# Autodesk Inventor assembly: ASY МОО 001 отстойник осветлитель
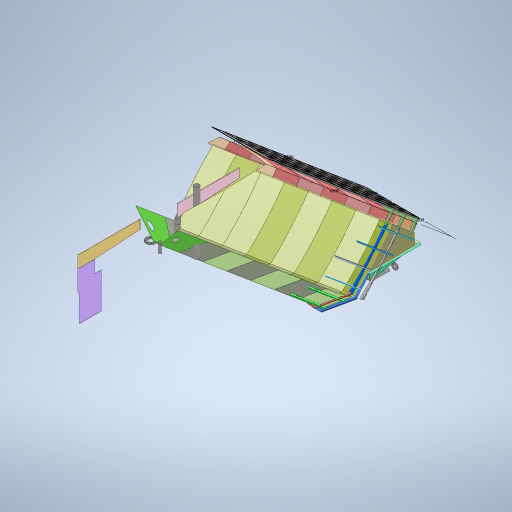
[picture p0: Inventor's stored thumbnail of the model, 512x512]
Saved by Autodesk Inventor 2024.2 (Build 282272000, 272)
## iProperties
Created: 2024-04-28
Part Number: ASY МОО 001 отстойник осветлитель
Document SubType Name: Weldment
Designer: admin
Weld Material: Welded Aluminum-6061
Mass: 1.58517e+06 g
Surface Area: 1.48953e+06 cm^2
Volume: 226523 cm^3
Density: 6.99781 g/cm^3
Author: admin
## Documents named in this file (42)
- C:\Users\admin\YandexDisk-badmisterfox\домашниий пк\Inventor\Manturovo\Manturovo_Se-clar\ASY МОО 001 отстойник осветлитель.iam
- C:\Users\admin\YandexDisk-badmisterfox\домашниий пк\Inventor\Manturovo\Manturovo_Se-clar\МОО 010 лист спина 1.ipt
- C:\Users\admin\YandexDisk-badmisterfox\домашниий пк\Inventor\Manturovo\Manturovo_Se-clar\Пример емкости.ipt
- C:\Users\admin\YandexDisk-badmisterfox\домашниий пк\Inventor\Manturovo\Manturovo_Se-clar\МОО 030 лист брюхо 1.ipt
- C:\Users\admin\YandexDisk-badmisterfox\домашниий пк\Inventor\Manturovo\Manturovo_Se-clar\МОО 040 шпангоут борт 1.ipt
- C:\Users\admin\YandexDisk-badmisterfox\домашниий пк\Inventor\Manturovo\Manturovo_Se-clar\МОО 041 шпангоут спина 1.ipt
- C:\Users\admin\YandexDisk-badmisterfox\домашниий пк\Inventor\Manturovo\Manturovo_Se-clar\Рама основания\ASY МОО 040 рама основания.iam
- C:\Users\admin\YandexDisk-badmisterfox\домашниий пк\Inventor\Manturovo\Manturovo_Se-clar\ASY МОО 060 ракета.iam
- C:\Users\admin\YandexDisk-badmisterfox\домашниий пк\Inventor\Manturovo\Manturovo_Se-clar\Content Center Files\en-US\ISO 5251 B 3D\ISO 5251 Bends 3D without straight ends(90 deg) DN80 2 2.ipt
- C:\Users\admin\YandexDisk-badmisterfox\домашниий пк\Inventor\Manturovo\Manturovo_Se-clar\Content Center Files\en-US\ISO 5251(1)\ISO 5251 Concentric reducers DN80 x DN65 3,2 3,2.ipt
- C:\Users\admin\YandexDisk-badmisterfox\домашниий пк\Inventor\Manturovo\Manturovo_Se-clar\ASY МОО 020 конус.iam
- C:\Users\admin\YandexDisk-badmisterfox\домашниий пк\Inventor\Manturovo\Manturovo_Se-clar\ракета\МОО 064 ракета труба.ipt
- C:\Users\admin\YandexDisk-badmisterfox\домашниий пк\Inventor\Manturovo\Manturovo_Se-clar\х_размеры МОО отстойник осветлитель Dummu.ipt
- C:\Users\admin\YandexDisk-badmisterfox\домашниий пк\Inventor\Manturovo\Manturovo_Se-clar\МОО 012 лист спина 2.ipt
- C:\Users\admin\YandexDisk-badmisterfox\домашниий пк\Inventor\Manturovo\Manturovo_Se-clar\Content Center Files\en-US\DIN EN 1092-1 01 - PN 25\DIN EN 1092-1 Plate Flange for Welding Type 01 - PN 25 80 x 88.9.ipt
- C:\Users\admin\YandexDisk-badmisterfox\домашниий пк\Inventor\Manturovo\Manturovo_Se-clar\МОО 011 лист борт.ipt
- C:\Users\admin\YandexDisk-badmisterfox\домашниий пк\Inventor\Manturovo\Manturovo_Se-clar\МОО 010 лист спина-бедро.ipt
- C:\Users\admin\YandexDisk-badmisterfox\домашниий пк\Inventor\Manturovo\Manturovo_Se-clar\МОО 011 лист борт левый борт бедро.ipt
- C:\Users\admin\YandexDisk-badmisterfox\домашниий пк\Inventor\Manturovo\Manturovo_Se-clar\МОО 011 лист борт правый борт бедро.ipt
- C:\Users\admin\YandexDisk-badmisterfox\домашниий пк\Inventor\Manturovo\Manturovo_Se-clar\МОО 014 лист спина-холка.ipt
- C:\Users\admin\YandexDisk-badmisterfox\домашниий пк\Inventor\Manturovo\Manturovo_Se-clar\МОО 032 лист брюхо-горло.ipt
- C:\Users\admin\YandexDisk-badmisterfox\домашниий пк\Inventor\Manturovo\Manturovo_Se-clar\МОО 035 лист борт.ipt
- C:\Users\admin\YandexDisk-badmisterfox\домашниий пк\Inventor\Manturovo\Manturovo_Se-clar\конус\МОО 051 гребень 1.ipt
- C:\Users\admin\YandexDisk-badmisterfox\домашниий пк\Inventor\Manturovo\Manturovo_Se-clar\конус\МОО 052 гребень 2.ipt
- C:\Users\admin\YandexDisk-badmisterfox\домашниий пк\Inventor\Manturovo\Manturovo_Se-clar\конус\МОО 053 морда 3.ipt
- C:\Users\admin\YandexDisk-badmisterfox\домашниий пк\Inventor\Manturovo\Manturovo_Se-clar\Content Center Files\en-US\ISO 5251 B 3D\ISO 5251 Bends 3D without straight ends(90 deg) DN150 11 11.ipt
- C:\Users\admin\YandexDisk-badmisterfox\домашниий пк\Inventor\Manturovo\Manturovo_Se-clar\Content Center Files\en-US\DIN EN 1092-1 01 - PN 25\DIN EN 1092-1 Plate Flange for Welding Type 01 - PN 25 150 x 168.3.ipt
- C:\Users\admin\YandexDisk-badmisterfox\домашниий пк\Inventor\Manturovo\Manturovo_Se-clar\МОО 061 труба верх 1.ipt
- C:\Users\admin\YandexDisk-badmisterfox\домашниий пк\Inventor\Manturovo\Manturovo_Se-clar\МОО 062 труба верх 2.ipt
- C:\Users\admin\YandexDisk-badmisterfox\домашниий пк\Inventor\Manturovo\Manturovo_Se-clar\МОО 063 труба верх 3.ipt
- C:\Users\admin\YandexDisk-badmisterfox\домашниий пк\Inventor\Manturovo\Manturovo_Se-clar\МОО 051 стрингер спина 1.ipt
- C:\Users\admin\YandexDisk-badmisterfox\домашниий пк\Inventor\Manturovo\Manturovo_Se-clar\МОО 053 стрингер борт 3.ipt
- C:\Users\admin\YandexDisk-badmisterfox\домашниий пк\Inventor\Manturovo\Manturovo_Se-clar\МОО 052 стрингер спина 22.ipt
- C:\Users\admin\YandexDisk-badmisterfox\домашниий пк\Inventor\Manturovo\Manturovo_Se-clar\МОО 054 стрингер борт 43.ipt
- C:\Users\admin\YandexDisk-badmisterfox\домашниий пк\Inventor\Manturovo\Manturovo_Se-clar\МОО 055 стрингер борт 52.ipt
- C:\Users\admin\YandexDisk-badmisterfox\домашниий пк\Inventor\Manturovo\Manturovo_Se-clar\МОО 056 стрингер борт 62.ipt
- C:\Users\admin\YandexDisk-badmisterfox\домашниий пк\Inventor\Manturovo\Manturovo_Se-clar\МОО 057 стрингер борт 7.ipt
- C:\Users\admin\YandexDisk-badmisterfox\домашниий пк\Inventor\Manturovo\Manturovo_Se-clar\МОО 042 шпангоут брюхо.ipt
- C:\Users\admin\YandexDisk-badmisterfox\домашниий пк\Inventor\Manturovo\Manturovo_Se-clar\МОО 025 лист борт холка.ipt
- C:\Users\admin\YandexDisk-badmisterfox\домашниий пк\Inventor\Manturovo\Manturovo_Se-clar\МОО 026 лист борт морда.ipt
- C:\Users\admin\YandexDisk-badmisterfox\домашниий пк\Inventor\Manturovo\Manturovo_Se-clar\Part1.ipt
- C:\Users\admin\YandexDisk-badmisterfox\домашниий пк\Inventor\Manturovo\Manturovo_Se-clar\стапель\ASY стапель.iam
## Components (82 placed, 43 different names)
1. Пример емкости:1 — Mate:1, Mate:2, Flush:2
2. х_размеры МОО отстойник осветлитель Dummu:1
3. ASY МОО 040 рама основания:1 [sub-assembly] — Flush:19, Flush:20, Flush:21
4. МОО 010 лист спина 1:1 — Flush:3, Rigid:11, Rigid:12
5. МОО 030 лист брюхо 1:1 — Mate:9, Rigid:18, Rigid:40
6. ASY МОО 060 ракета:1 [sub-assembly] — Flush:23, Rigid:10
7. ISO 5251 Bends 3D without straight ends(90 deg) DN80 2:1 — Rigid:2, Rigid:3
8. ISO 5251 Concentric reducers DN80 x DN65 3,2:1 — Rigid:2, Rigid:10
9. ASY МОО 020 конус:1 [sub-assembly] — Flush:22, Mate:16, Flush:28, Mate:31, Mate:36, Mate:54, Mate:57
10. МОО 064 ракета труба:1 — Rigid:3, Cylindrical:1
11. МОО 010 лист спина 1:2 — Rigid:11, Tangent:1, Tangent:3, Rigid:37
12. МОО 010 лист спина 1:3 — Flush:24, Rigid:12, Mate:19, Mate:22, Rigid:30, Mate:31, Flush:44, Tangent:8, Tangent:9
13. МОО 012 лист спина 2:1 — Mate:15, Mate:16, Flush:27, Mate:19, Mate:22
14. DIN EN 1092-1 Plate Flange for Welding Type 01 - PN 25 80 x 88.9:1 — Flush:25, Flush:26, Mate:18, Cylindrical:1
15. МОО 011 лист борт:1 — Flush:30, Tangent:1, Rigid:35, Mate:37
16. МОО 030 лист брюхо 1:2 — Rigid:18, Rigid:53
17. МОО 010 лист спина-бедро:1 — Mate:24, Rigid:30, Flush:42, Tangent:6, Flush:43, Tangent:7
18. МОО 011 лист борт левый борт бедро:1 — Flush:41, Flush:42, Tangent:6
19. МОО 011 лист борт правый борт бедро:1 — Mate:30, Flush:43, Tangent:7
20. МОО 011 лист борт:7 — Rigid:35, Rigid:36
21. МОО 011 лист борт:8 — Rigid:36, Rigid:49
22. МОО 010 лист спина 1:5 — Rigid:37, Rigid:38
23. МОО 010 лист спина 1:6 — Rigid:38, Rigid:39
24. МОО 014 лист спина-холка:1 — Rigid:39
25. МОО 030 лист брюхо 1:4 — Rigid:40, Rigid:47
26. МОО 032 лист брюхо-горло:1 — Rigid:48, Mate:52, Mate:53, Rigid:54, Rigid:61
27. МОО 030 лист брюхо 1:5 — Rigid:45, Rigid:47
28. МОО 030 лист брюхо 1:6 — Rigid:45, Rigid:48
29. МОО 011 лист борт:9 — Rigid:49, Rigid:50
30. МОО 024 лист борт — Rigid:50, Rigid:113
31. МОО 035 лист борт:1 — Mate:36, Flush:47, Tangent:8, Mate:37, Mate:55
32. МОО 051 гребень 1:1 — Mate:50, Mate:56, Flush:48
33. МОО 052 гребень 2:1 — Rigid:56
34. МОО 053 морда 3:1 — Mate:51, Mate:52, Rigid:52, Mate:53, Mate:56, Mate:59, Flush:49
35. МОО 053 морда 3:2 — Rigid:52, Flush:48
36. МОО 030 лист брюхо 1:7 — Mate:54, Mate:55, Rigid:53
37. DIN EN 1092-1 Plate Flange for Welding Type 01 - PN 25 80 x 88.9:2 — Rigid:54, Rigid:62
38. МОО 051 гребень 1:2 — Rigid:56
39. МОО 052 гребень 2:2 — Mate:59, Flush:49
40. DIN EN 1092-1 Plate Flange for Welding Type 01 - PN 25 150 x 168.3:1 — Rotational:1
41. МОО 061 труба верх 1:1 — Rotational:1, Rigid:59
42. ISO 5251 Bends 3D without straight ends(90 deg) DN150 11:1 — Rigid:59
43. МОО 062 труба верх 2:1
44. DIN EN 1092-1 Plate Flange for Welding Type 01 - PN 25 150 x 168.3:2 — Rigid:61
45. МОО 063 труба верх 3:1 — Rigid:62
46. МОО 011 лист борт:11
47. МОО 011 лист борт:12
48. МОО 011 лист борт:13
49. МОО 011 лист борт:14
50. МОО 011 лист борт:15 — Rigid:67
51. МОО 035 лист борт:2 — Rigid:67, Mate:57, Mate:58, Tangent:9
52. МОО 040 шпангоут борт 1:2 — Rigid:74, Rigid:128, Rigid:129
53. МОО 041 шпангоут спина 1:3 — Rigid:25, Rigid:74, Rigid:91, Rigid:93
54. МОО 056 стрингер борт 6:2
55. МОО 055 стрингер борт 5:2
56. МОО 054 стрингер борт 4:2 — Rigid:129
57. МОО 053 стрингер борт 3:2 — Rigid:128
58. МОО 052 стрингер спина 2:2 — Rigid:93
59. МОО 051 стрингер спина 1:2 — Rigid:91
60. МОО 051 стрингер спина 1:1 — Rigid:90
61. МОО 025 лист борт холка:1 — Rigid:113, Rigid:114
62. МОО 026 лист борт морда:1 — Rigid:114
63. Part1:1
64. МОО 041 шпангоут спина 1:26 — Rigid:116, Rigid:121, Rigid:130, Rigid:131
65. МОО 041 шпангоут спина 1:27 — Rigid:116
66. МОО 041 шпангоут спина 1:28 — Rigid:131
67. МОО 041 шпангоут спина 1:29 — Mate:62, Flush:53
68. МОО 040 шпангоут борт 1:3 — Rigid:121
69. МОО 052 стрингер спина 2:1 — Rigid:92
70. МОО 056 стрингер борт 6:1 — Rigid:125
71. МОО 053 стрингер борт 3:1 — Rigid:122
72. МОО 054 стрингер борт 4:1 — Rigid:123
73. МОО 055 стрингер борт 5:1 — Rigid:124
74. МОО 040 шпангоут борт 1:1 — Rigid:72, Rigid:122, Rigid:123, Flush:51, Flush:52, Rigid:124, Rigid:125, Mate:61
75. МОО 041 шпангоут спина БАЗА 1:2 — Flush:12, Tangent:3, Rigid:25, Flush:44, Rigid:72, Rigid:90, Rigid:92, Rigid:130
76. ASY стапель:1 [sub-assembly] — Mate:62, Flush:53, Mate:63
77. МОО 042 шпангоут брюхо:2 — Rigid:111, Rigid:112, Rigid:127
78. МОО 042 шпангоут брюхо:1 — Rigid:110, Flush:51, Flush:52, Rigid:126, Mate:61, Rigid:127
79. МОО 057 стрингер борт 7:3 — Rigid:111
80. МОО 057 стрингер борт 7:4 — Rigid:112
81. МОО 057 стрингер борт 7:1 — Rigid:126
82. МОО 057 стрингер борт 7:2 — Rigid:110
## Relationships (113: WeldJoint 55, Mate 26, Flush 24, Tangent 6, CylindricalJoint 1, RevoluteJoint 1)
- Mate:1: Пример емкости:1
- Mate:2: Пример емкости:1
- Flush:2: Пример емкости:1
- Flush:3: МОО 010 лист спина 1:1
- Mate:9: МОО 030 лист брюхо 1:1
- Flush:12: МОО 041 шпангоут спина БАЗА 1:2
- Rigid:2 [WeldJoint]: ISO 5251 Bends 3D without straight ends(90 deg) DN80 2:1 ↔ ISO 5251 Concentric reducers DN80 x DN65 3,2:1
- Rigid:3 [WeldJoint]: ISO 5251 Bends 3D without straight ends(90 deg) DN80 2:1 ↔ МОО 064 ракета труба:1
- Flush:19 (-250 mm): ASY МОО 040 рама основания:1
- Flush:20: ASY МОО 040 рама основания:1
- Flush:21: ASY МОО 040 рама основания:1
- Flush:22: ASY МОО 020 конус:1
- Flush:23: ASY МОО 060 ракета:1
- Mate:15: МОО 012 лист спина 2:1
- Flush:24: МОО 010 лист спина 1:3
- Mate:16: ASY МОО 020 конус:1 ↔ МОО 012 лист спина 2:1
- Flush:25: DIN EN 1092-1 Plate Flange for Welding Type 01 - PN 25 80 x 88.9:1
- Flush:26: DIN EN 1092-1 Plate Flange for Welding Type 01 - PN 25 80 x 88.9:1
- Mate:18 (120 mm): DIN EN 1092-1 Plate Flange for Welding Type 01 - PN 25 80 x 88.9:1
- Rigid:10 [WeldJoint] (-20 mm): ASY МОО 060 ракета:1 ↔ ISO 5251 Concentric reducers DN80 x DN65 3,2:1
- Cylindrical:1: МОО 064 ракета труба:1 ↔ DIN EN 1092-1 Plate Flange for Welding Type 01 - PN 25 80 x 88.9:1
- Flush:27 (15 mm): МОО 012 лист спина 2:1
- Flush:28: ASY МОО 020 конус:1
- Rigid:11 [WeldJoint]: МОО 010 лист спина 1:1 ↔ МОО 010 лист спина 1:2
- Rigid:12 [WeldJoint]: МОО 010 лист спина 1:1 ↔ МОО 010 лист спина 1:3
- Mate:19 (910 mm): МОО 010 лист спина 1:3 ↔ МОО 012 лист спина 2:1
- Flush:30: МОО 011 лист борт:1
- Tangent:1: МОО 010 лист спина 1:2 ↔ МОО 011 лист борт:1
- Tangent:3: МОО 010 лист спина 1:2 ↔ МОО 041 шпангоут спина БАЗА 1:2
- Mate:22 (47 mm): МОО 010 лист спина 1:3 ↔ МОО 012 лист спина 2:1
- Rigid:18 [WeldJoint]: МОО 030 лист брюхо 1:1 ↔ МОО 030 лист брюхо 1:2
- Rigid:25 [WeldJoint] (-50 mm): МОО 041 шпангоут спина 1:3 ↔ МОО 041 шпангоут спина БАЗА 1:2
- Mate:24: МОО 010 лист спина-бедро:1
- Rigid:30 [WeldJoint]: МОО 010 лист спина 1:3 ↔ МОО 010 лист спина-бедро:1
- Flush:41: МОО 011 лист борт левый борт бедро:1
- Flush:42: МОО 010 лист спина-бедро:1 ↔ МОО 011 лист борт левый борт бедро:1
- Tangent:6: МОО 010 лист спина-бедро:1 ↔ МОО 011 лист борт левый борт бедро:1
- Mate:30: МОО 011 лист борт правый борт бедро:1
- Flush:43: МОО 010 лист спина-бедро:1 ↔ МОО 011 лист борт правый борт бедро:1
- Tangent:7: МОО 010 лист спина-бедро:1 ↔ МОО 011 лист борт правый борт бедро:1
- Rigid:35 [WeldJoint]: МОО 011 лист борт:1 ↔ МОО 011 лист борт:7
- Rigid:36 [WeldJoint]: МОО 011 лист борт:7 ↔ МОО 011 лист борт:8
- Rigid:37 [WeldJoint]: МОО 010 лист спина 1:2 ↔ МОО 010 лист спина 1:5
- Rigid:38 [WeldJoint]: МОО 010 лист спина 1:5 ↔ МОО 010 лист спина 1:6
- Rigid:39 [WeldJoint]: МОО 010 лист спина 1:6 ↔ МОО 014 лист спина-холка:1
- Mate:31: ASY МОО 020 конус:1 ↔ МОО 010 лист спина 1:3
- Rigid:40 [WeldJoint]: МОО 030 лист брюхо 1:1 ↔ МОО 030 лист брюхо 1:4
- Flush:44 (-250 mm): МОО 010 лист спина 1:3 ↔ МОО 041 шпангоут спина БАЗА 1:2
- Rigid:45 [WeldJoint]: МОО 030 лист брюхо 1:5 ↔ МОО 030 лист брюхо 1:6
- Rigid:47 [WeldJoint]: МОО 030 лист брюхо 1:4 ↔ МОО 030 лист брюхо 1:5
- Rigid:48 [WeldJoint]: МОО 032 лист брюхо-горло:1 ↔ МОО 030 лист брюхо 1:6
- Rigid:49 [WeldJoint]: МОО 011 лист борт:8 ↔ МОО 011 лист борт:9
- Rigid:50 [WeldJoint]: МОО 011 лист борт:9 ↔ МОО 024 лист борт
- Mate:36: ASY МОО 020 конус:1 ↔ МОО 035 лист борт:1
- Flush:47: МОО 035 лист борт:1
- Tangent:8: МОО 010 лист спина 1:3 ↔ МОО 035 лист борт:1
- Mate:37: МОО 011 лист борт:1 ↔ МОО 035 лист борт:1
- Mate:50 (200 mm): МОО 051 гребень 1:1
- Mate:51: МОО 053 морда 3:1
- Mate:52: МОО 032 лист брюхо-горло:1 ↔ МОО 053 морда 3:1
- Rigid:52 [WeldJoint]: МОО 053 морда 3:1 ↔ МОО 053 морда 3:2
- Mate:53 (-10 mm): МОО 032 лист брюхо-горло:1 ↔ МОО 053 морда 3:1
- Mate:54: ASY МОО 020 конус:1 ↔ МОО 030 лист брюхо 1:7
- Mate:55: МОО 035 лист борт:1 ↔ МОО 030 лист брюхо 1:7
- Rigid:53 [WeldJoint]: МОО 030 лист брюхо 1:2 ↔ МОО 030 лист брюхо 1:7
- Mate:56 (450 mm): МОО 051 гребень 1:1 ↔ МОО 053 морда 3:1
- Rigid:54 [WeldJoint] (200 mm): МОО 032 лист брюхо-горло:1 ↔ DIN EN 1092-1 Plate Flange for Welding Type 01 - PN 25 80 x 88.9:2
- Flush:48 (-200 mm): МОО 051 гребень 1:1 ↔ МОО 053 морда 3:2
- Rigid:56 [WeldJoint]: МОО 052 гребень 2:1 ↔ МОО 051 гребень 1:2
- Rotational:1 [RevoluteJoint]: DIN EN 1092-1 Plate Flange for Welding Type 01 - PN 25 150 x 168.3:1 ↔ МОО 061 труба верх 1:1
- Rigid:59 [WeldJoint]: МОО 061 труба верх 1:1 ↔ ISO 5251 Bends 3D without straight ends(90 deg) DN150 11:1
- Rigid:61 [WeldJoint] (300 mm): МОО 032 лист брюхо-горло:1 ↔ DIN EN 1092-1 Plate Flange for Welding Type 01 - PN 25 150 x 168.3:2
- Rigid:62 [WeldJoint]: DIN EN 1092-1 Plate Flange for Welding Type 01 - PN 25 80 x 88.9:2 ↔ МОО 063 труба верх 3:1
- [WeldJoint]: МОО 011 лист борт:11 ↔ МОО 011 лист борт:12
- [WeldJoint]: МОО 011 лист борт:12 ↔ МОО 011 лист борт:13
- [WeldJoint]: МОО 011 лист борт:13 ↔ МОО 011 лист борт:14
- [WeldJoint]: МОО 011 лист борт:14 ↔ МОО 011 лист борт:15
- Rigid:67 [WeldJoint]: МОО 011 лист борт:15 ↔ МОО 035 лист борт:2
- Mate:57: ASY МОО 020 конус:1 ↔ МОО 035 лист борт:2
- Mate:58: МОО 035 лист борт:2
- Tangent:9: МОО 010 лист спина 1:3 ↔ МОО 035 лист борт:2
- Rigid:72 [WeldJoint] (-50 mm): МОО 040 шпангоут борт 1:1 ↔ МОО 041 шпангоут спина БАЗА 1:2
- Rigid:74 [WeldJoint] (-50 mm): МОО 040 шпангоут борт 1:2 ↔ МОО 041 шпангоут спина 1:3
- Rigid:90 [WeldJoint] (2 mm): МОО 051 стрингер спина 1:1 ↔ МОО 041 шпангоут спина БАЗА 1:2
- Rigid:91 [WeldJoint] (2 mm): МОО 041 шпангоут спина 1:3 ↔ МОО 051 стрингер спина 1:2
- Rigid:92 [WeldJoint] (2 mm): МОО 052 стрингер спина 2:1 ↔ МОО 041 шпангоут спина БАЗА 1:2
- Rigid:93 [WeldJoint] (2 mm): МОО 041 шпангоут спина 1:3 ↔ МОО 052 стрингер спина 2:2
- Rigid:110 [WeldJoint] (2 mm): МОО 042 шпангоут брюхо:1 ↔ МОО 057 стрингер борт 7:2
- Rigid:111 [WeldJoint] (2 mm): МОО 042 шпангоут брюхо:2 ↔ МОО 057 стрингер борт 7:3
- Rigid:112 [WeldJoint] (2 mm): МОО 042 шпангоут брюхо:2 ↔ МОО 057 стрингер борт 7:4
- Rigid:113 [WeldJoint]: МОО 024 лист борт ↔ МОО 025 лист борт холка:1
- Rigid:114 [WeldJoint]: МОО 025 лист борт холка:1 ↔ МОО 026 лист борт морда:1
- Rigid:116 [WeldJoint] (50 mm): МОО 041 шпангоут спина 1:26 ↔ МОО 041 шпангоут спина 1:27
- [WeldJoint] (50 mm): МОО 041 шпангоут спина 1:28 ↔ МОО 041 шпангоут спина 1:29
- Rigid:121 [WeldJoint] (-50 mm): МОО 041 шпангоут спина 1:26 ↔ МОО 040 шпангоут борт 1:3
- Rigid:122 [WeldJoint] (2 mm): МОО 053 стрингер борт 3:1 ↔ МОО 040 шпангоут борт 1:1
- Rigid:123 [WeldJoint] (2 mm): МОО 054 стрингер борт 4:1 ↔ МОО 040 шпангоут борт 1:1
- Mate:59 (-450 mm): МОО 053 морда 3:1 ↔ МОО 052 гребень 2:2
- Flush:49: МОО 053 морда 3:1 ↔ МОО 052 гребень 2:2
- Flush:51: МОО 040 шпангоут борт 1:1 ↔ МОО 042 шпангоут брюхо:1
- Flush:52: МОО 040 шпангоут борт 1:1 ↔ МОО 042 шпангоут брюхо:1
- Rigid:124 [WeldJoint] (2 mm): МОО 055 стрингер борт 5:1 ↔ МОО 040 шпангоут борт 1:1
- Rigid:125 [WeldJoint]: МОО 056 стрингер борт 6:1 ↔ МОО 040 шпангоут борт 1:1
- Rigid:126 [WeldJoint] (2 mm): МОО 042 шпангоут брюхо:1 ↔ МОО 057 стрингер борт 7:1
- Mate:61: МОО 040 шпангоут борт 1:1 ↔ МОО 042 шпангоут брюхо:1
- Mate:62: МОО 041 шпангоут спина 1:29 ↔ ASY стапель:1
- Flush:53: МОО 041 шпангоут спина 1:29 ↔ ASY стапель:1
- Mate:63: ASY стапель:1
- Rigid:127 [WeldJoint] (-50 mm): МОО 042 шпангоут брюхо:2 ↔ МОО 042 шпангоут брюхо:1
- Rigid:128 [WeldJoint] (2 mm): МОО 040 шпангоут борт 1:2 ↔ МОО 053 стрингер борт 3:2
- Rigid:129 [WeldJoint] (2 mm): МОО 040 шпангоут борт 1:2 ↔ МОО 054 стрингер борт 4:2
- Rigid:130 [WeldJoint] (-500 mm): МОО 041 шпангоут спина 1:26 ↔ МОО 041 шпангоут спина БАЗА 1:2
- Rigid:131 [WeldJoint] (-500 mm): МОО 041 шпангоут спина 1:26 ↔ МОО 041 шпангоут спина 1:28
## Named parameters: Бак_нахлест_фланца = 25 mm, d230_d194 = 0 mm, d231_d195 = 0 mm, d232_d160 = 0 mm, d233_d161 = 0 mm, d322_d320 = 50 mm
